# Autodesk Inventor assembly: BatteryHolderAssembly
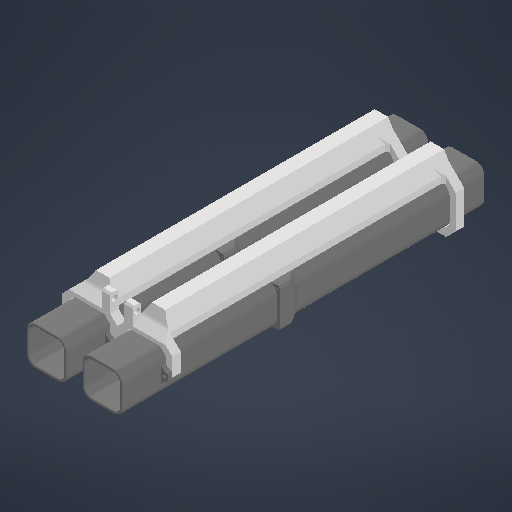
[picture p0: Inventor's stored thumbnail of the model, 512x512]
Saved by Autodesk Inventor 2026.1 (Build 301233000, 233)
## iProperties
Created: 2026-06-27
Part Number: BatteryHolderAssembly
Document SubType Name: Assembly
Designer: Brynjar
Author: Brynjar
## Documents named in this file (3)
- C:\Users\brynj\Documents\Inventor\Workspaces\Project S.Ó.F.I\#2\BatteryHolderAssembly.iam
- C:\Users\brynj\Documents\Inventor\Workspaces\Project S.Ó.F.I\#2\BatteryHolderBracket.ipt
- C:\Users\brynj\Documents\Inventor\Workspaces\Project S.Ó.F.I\#2\BatteryHolder.ipt
## Components (3 placed, 2 different names)
1. BatteryHolderBracket:1 — Rotational:1, Rotational:2, Rotational:3, Rotational:4
2. BatteryHolder:1 — Rotational:1, Rotational:2
3. BatteryHolder:2 — Rotational:3, Rotational:4
## Relationships (4: RevoluteJoint 4)
- Rotational:1 [RevoluteJoint]: BatteryHolderBracket:1 ↔ BatteryHolder:1
- Rotational:2 [RevoluteJoint]: BatteryHolderBracket:1 ↔ BatteryHolder:1
- Rotational:3 [RevoluteJoint]: BatteryHolderBracket:1 ↔ BatteryHolder:2
- Rotational:4 [RevoluteJoint]: BatteryHolderBracket:1 ↔ BatteryHolder:2
